# Autodesk Inventor assembly: simpleGBFull
Saved by Autodesk Inventor 2015 (Build 190159000, 159)
## iProperties
Created: 2015-01-30
Part Number: simpleGBFull
Document SubType Name: Assembly
Designer: Kingbob26
Author: Kingbob26
## Documents named in this file (5)
- C:\Users\Kingbob26\Documents\GitHub\2015CAD\actualWheelBase\Drive Base\Parts\simpleGBFull.iam
- C:\Users\Kingbob26\Documents\GitHub\2015CAD\wheelBase\CIM Motor SW.ipt
- C:\Users\Kingbob26\Documents\GitHub\2015CAD\wheelBase\gearBoxSimple\simpleGBHousing.ipt
- C:\Users\Kingbob26\Documents\GitHub\2015CAD\wheelBase\gearBoxSimple\simpleGBMount.ipt
- C:\Users\Kingbob26\Documents\GitHub\2015CAD\wheelBase\gearBoxSimple\simpleGBStopBlockSmallCylindrical.ipt
## Components (4 placed, 4 different names)
1. CIM Motor SW:1
2. simpleGBHousing:1
3. simpleGBMount:1
4. simpleGBStopBlockSmallCylindrical:1
## Relationships (7: Mate 7)
- [Mate]: simpleGBHousing:1 ↔ simpleGBMount:1
- [Mate]: simpleGBHousing:1 ↔ simpleGBMount:1
- [Mate]: simpleGBHousing:1 ↔ simpleGBMount:1
- [Mate]: simpleGBHousing:1 ↔ simpleGBStopBlockSmallCylindrical:1
- [Mate]: simpleGBHousing:1 ↔ simpleGBStopBlockSmallCylindrical:1
- [Mate]: CIM Motor SW:1 ↔ simpleGBHousing:1
- [Mate]: CIM Motor SW:1 ↔ simpleGBHousing:1
